# Autodesk Inventor assembly: NEUROPIXELS GEN 1 PROBE ASSY
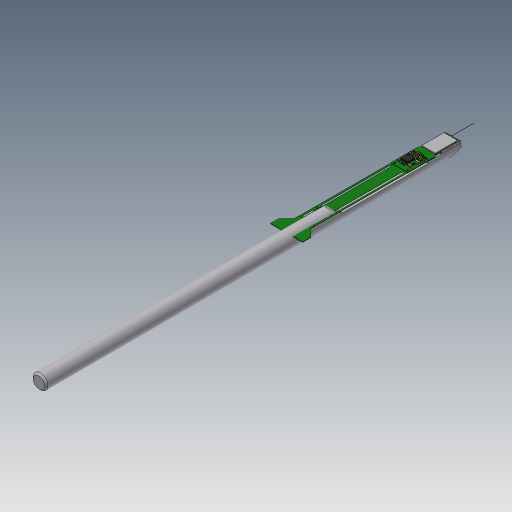
[picture p0: Inventor's stored thumbnail of the model, 512x512]
Saved by Autodesk Inventor 2023.4 (Build 274418000, 418)
## iProperties
RuleStatus: InUse
AfterDocSave0: file://Part Number Cleaner
Created: 2019-07-02
Vendor: HHMI: JRC - ID&F
Document SubType Name: Assembly
Designer: arnoldj
DESIGN DEPARTMENT: HHMI: JRC - ID&F
LAB/DEPT: A. LEE (LAB)
ALTERED ITEM PART NUMBER: N/A
ALTERED ITEM VENDOR: N/A
ALTERED ITEM DESCRIPTION: N/A
Author: arnoldj
Revision Number: 0
## Documents named in this file (5)
- C:\_WORKSPACE\DATA\PROJECTS\PROBE MOUNTS\MCAD\NEUROPIXELS GEN 1 PROBE ASSY.iam
- C:\_WORKSPACE\DATA\PROJECTS\PROBE MOUNTS\MCAD\NEUROPIXELS DOVE TAIL PROBE HOLDER.ipt
- C:\_WORKSPACE\DATA\PROJECTS\PROBE MOUNTS\MCAD\NP2_FLEX_00-01.ipt
- C:\_WORKSPACE\DATA\PROJECTS\PROBE MOUNTS\MCAD\NEUROPIXELS DOVE TAIL MOUNT.ipt
- C:\_WORKSPACE\DATA\COMMON\Misumi\MISUMI SSHHI-SUS-M2.5-2.5.ipt
## Components (4 placed, 4 different names)
1. NEUROPIXELS DOVE TAIL PROBE HOLDER:1 — Mate:1, Mate:2, Flush:1, Mate:8
2. NEUROPIXELS DOVE TAIL MOUNT:1 — Mate:1, Mate:2, Flush:1, Mate:6, Flush:5, Mate:7
3. NP2_FLEX_00-01:1 — Mate:6, Flush:5, Flush:6
4. MISUMI SSHHI-SUS-M2.5-2.5:1 — Mate:7, Mate:8
## Relationships (8: Mate 5, Flush 3)
- Mate:1: NEUROPIXELS DOVE TAIL PROBE HOLDER:1 ↔ NEUROPIXELS DOVE TAIL MOUNT:1
- Mate:2: NEUROPIXELS DOVE TAIL PROBE HOLDER:1 ↔ NEUROPIXELS DOVE TAIL MOUNT:1
- Flush:1: NEUROPIXELS DOVE TAIL PROBE HOLDER:1 ↔ NEUROPIXELS DOVE TAIL MOUNT:1
- Mate:6: NEUROPIXELS DOVE TAIL MOUNT:1 ↔ NP2_FLEX_00-01:1
- Flush:5: NEUROPIXELS DOVE TAIL MOUNT:1 ↔ NP2_FLEX_00-01:1
- Flush:6 (0.3556 mm): NP2_FLEX_00-01:1
- Mate:7: NEUROPIXELS DOVE TAIL MOUNT:1 ↔ MISUMI SSHHI-SUS-M2.5-2.5:1
- Mate:8: NEUROPIXELS DOVE TAIL PROBE HOLDER:1 ↔ MISUMI SSHHI-SUS-M2.5-2.5:1
